# Autodesk Inventor assembly: turntable + gear
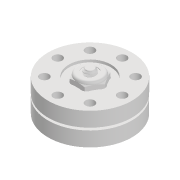
[picture p0: Inventor's stored thumbnail of the model, 180x180]
Saved by Autodesk Inventor 2020 (Build 240168000, 168)
## iProperties
Created: 2020-01-01
Part Number: turntable + gear
Document SubType Name: Assembly
Designer: ball
Author: ball
## Documents named in this file (3)
- C:\FTC\FTC8863CAD\2019 Robot\Collection\turntable + gear.iam
- C:\FTC\FTC8863CAD\Actobotics\545 parts\545364 assembly.ipt
- C:\FTC\FTC8863CAD\Actobotics\615 parts\615190.ipt
## Components (2 placed, 2 different names)
1. 545364 assembly:1 — Mate:1, Mate:2, Mate:3
2. 615190:1 — Mate:1, Mate:2, Mate:3
## Relationships (3: Mate 3)
- Mate:1: 545364 assembly:1 ↔ 615190:1
- Mate:2: 545364 assembly:1 ↔ 615190:1
- Mate:3: 545364 assembly:1 ↔ 615190:1
